# Autodesk Inventor assembly: pelvis_w_motor1
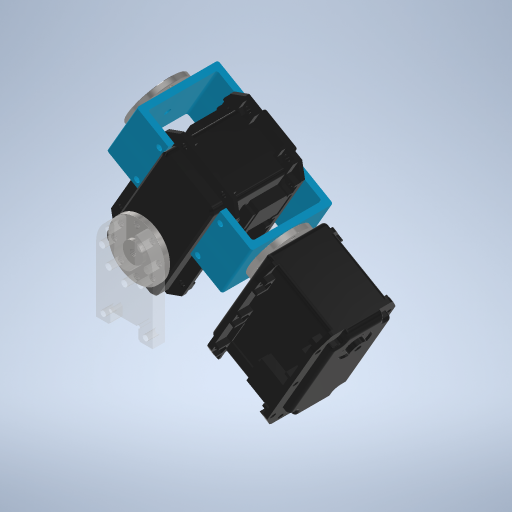
[picture p0: Inventor's stored thumbnail of the model, 512x512]
Saved by Autodesk Inventor 2024 (Build 280153000, 153)
## iProperties
Created: 2024-09-14
Part Number: pelvis_w_motor1
Document SubType Name: Assembly
Designer: jmha0
Author: jmha0
## Documents named in this file (9)
- C:\Users\jmha0\OneDrive\바탕 화면\19th_intern_hjm_fight_robot\부품\Lower_Body\pelvis_w_motor\pelvis_w_motor_fin1.iam
- C:\Users\jmha0\OneDrive\바탕 화면\19th_intern_hjm_fight_robot\부품\Lower_Body\pelvis_w_motor\frame_knee_to_pelvis1.ipt
- C:\Users\jmha0\OneDrive\바탕 화면\19th_intern_hjm_fight_robot\부품\hardware\ROBOTIS(Inventor 2024 ver.)\다이나믹셀\MX-106T+idle.ipt.iam
- C:\Users\jmha0\OneDrive\바탕 화면\19th_intern_hjm_fight_robot\부품\hardware\ROBOTIS(Inventor 2024 ver.)\다이나믹셀\MX-64T.ipt
- C:\Users\jmha0\OneDrive\바탕 화면\19th_intern_hjm_fight_robot\부품\hardware\ROBOTIS(Inventor 2024 ver.)\아이들러\64아이들러.iam
- C:\Users\jmha0\OneDrive\바탕 화면\19th_intern_hjm_fight_robot\부품\hardware\ROBOTIS(Inventor 2024 ver.)\혼\64-106Horn.ipt
- C:\Users\jmha0\OneDrive\바탕 화면\19th_intern_hjm_fight_robot\부품\Lower_Body\pelvis_w_motor\3D_pelvis2.ipt
- C:\Users\jmha0\OneDrive\바탕 화면\19th_intern_hjm_fight_robot\부품\Lower_Body\pelvis_w_motor\3D_pelvis1.ipt
- MX-106T+idle.ipt
## Components (9 placed, 7 different names)
1. frame_knee_to_pelvis1:1 — 삽입:2, 삽입:3, 삽입:4, 삽입:5, 삽입:6, 삽입:7, 각도:1, 각도:3, 각도:4
2. MX-106T+idle.ipt:1 [sub-assembly] — 삽입:1, 삽입:12, 삽입:13, 삽입:14, 삽입:15, 삽입:16, 삽입:17, 메이트:1, 각도:2, 각도:4
3. MX-64T:1 — 삽입:18, 각도:2
4. 64아이들러:1 [sub-assembly] — 삽입:21
5. 64-106Horn:1 — 삽입:1, 삽입:2, 삽입:3, 삽입:4, 삽입:5, 삽입:6, 삽입:7
6. frame_knee_to_pelvis1:2 — 메이트:1, 각도:1, 각도:3
7. 3D_pelvis2:1 — 삽입:15, 삽입:16, 삽입:17, 삽입:19, 삽입:20
8. 3D_pelvis1:1 — 삽입:12, 삽입:13, 삽입:14, 삽입:21
9. 64-106Horn:2 — 삽입:18, 삽입:19, 삽입:20
## Relationships (22: Insert 17, Angle 4, Mate 1)
- 삽입:1 [Insert] (0.1 mm): MX-106T+idle.ipt:1 ↔ 64-106Horn:1
- 삽입:2 [Insert]: frame_knee_to_pelvis1:1 ↔ 64-106Horn:1
- 삽입:3 [Insert]: frame_knee_to_pelvis1:1 ↔ 64-106Horn:1
- 삽입:4 [Insert]: frame_knee_to_pelvis1:1 ↔ 64-106Horn:1
- 삽입:5 [Insert]: frame_knee_to_pelvis1:1 ↔ 64-106Horn:1
- 삽입:6 [Insert]: frame_knee_to_pelvis1:1 ↔ 64-106Horn:1
- 삽입:7 [Insert]: frame_knee_to_pelvis1:1 ↔ 64-106Horn:1
- 삽입:12 [Insert]: MX-106T+idle.ipt:1 ↔ 3D_pelvis1:1
- 삽입:13 [Insert]: MX-106T+idle.ipt:1 ↔ 3D_pelvis1:1
- 삽입:14 [Insert]: MX-106T+idle.ipt:1 ↔ 3D_pelvis1:1
- 삽입:15 [Insert]: MX-106T+idle.ipt:1 ↔ 3D_pelvis2:1
- 삽입:16 [Insert]: MX-106T+idle.ipt:1 ↔ 3D_pelvis2:1
- 삽입:17 [Insert]: MX-106T+idle.ipt:1 ↔ 3D_pelvis2:1
- 삽입:18 [Insert] (0.1 mm): MX-64T:1 ↔ 64-106Horn:2
- 삽입:19 [Insert]: 3D_pelvis2:1 ↔ 64-106Horn:2
- 삽입:20 [Insert]: 3D_pelvis2:1 ↔ 64-106Horn:2
- 삽입:21 [Insert]: 64아이들러:1 ↔ 3D_pelvis1:1
- 메이트:1 [Mate]: MX-106T+idle.ipt:1 ↔ frame_knee_to_pelvis1:2
- 각도:1 [Angle] (0 deg): frame_knee_to_pelvis1:1 ↔ frame_knee_to_pelvis1:2
- 각도:2 [Angle] (0 deg): MX-106T+idle.ipt:1 ↔ MX-64T:1
- 각도:3 [Angle] (0 deg): frame_knee_to_pelvis1:1 ↔ frame_knee_to_pelvis1:2
- 각도:4 [Angle] (30 deg): frame_knee_to_pelvis1:1 ↔ MX-106T+idle.ipt:1
